# Autodesk Inventor assembly: TWambatDrive
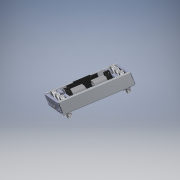
[picture p0: Inventor's stored thumbnail of the model, 180x180]
Saved by Autodesk Inventor 2019 (Build 230136000, 136)
## iProperties
Created: 2019-12-10
Part Number: TWambatDrive
Document SubType Name: Assembly
Designer: james
Author: james
## Documents named in this file (5)
- F:\JimsRobot\FIRSTRobots\Design\TWambat\TWambatDrive.iam
- F:\JimsRobot\FIRSTRobots\Design\TWambat\TWambat Side.iam
- F:\JimsRobot\FIRSTRobots\Design\TWambat\BackBatteryPlate.ipt
- F:\JimsRobot\FIRSTRobots\Design\TWambat\TWambat End Sheet.ipt
- F:\JimsRobot\FIRSTRobots\Design\TWambat\TWambat Front Sheet.ipt
## Components (6 placed, 4 different names)
1. TWambat Side:1 [sub-assembly] — Mate:1, Mate:2, Mate:3, Mate:13, Mate:14, Mate:15
2. BackBatteryPlate:1 — Mate:4, Mate:5, Mate:6, Mate:7, Mate:8, Mate:9
3. TWambat End Sheet:1 — Mate:1, Mate:2, Mate:3, Mate:4, Mate:5, Mate:6
4. TWambat End Sheet:2 — Mate:7, Mate:8, Mate:9, Mate:10, Mate:11, Mate:12
5. TWambat Side:2 [sub-assembly] — Mate:10, Mate:11, Mate:12
6. TWambat Front Sheet:1 — Mate:13, Mate:14, Mate:15
## Relationships (15: Mate 15)
- Mate:1: TWambat Side:1 ↔ TWambat End Sheet:1
- Mate:2: TWambat Side:1 ↔ TWambat End Sheet:1
- Mate:3: TWambat Side:1 ↔ TWambat End Sheet:1
- Mate:4: BackBatteryPlate:1 ↔ TWambat End Sheet:1
- Mate:5: BackBatteryPlate:1 ↔ TWambat End Sheet:1
- Mate:6: BackBatteryPlate:1 ↔ TWambat End Sheet:1
- Mate:7: BackBatteryPlate:1 ↔ TWambat End Sheet:2
- Mate:8: BackBatteryPlate:1 ↔ TWambat End Sheet:2
- Mate:9: BackBatteryPlate:1 ↔ TWambat End Sheet:2
- Mate:10: TWambat End Sheet:2 ↔ TWambat Side:2
- Mate:11: TWambat End Sheet:2 ↔ TWambat Side:2
- Mate:12: TWambat End Sheet:2 ↔ TWambat Side:2
- Mate:13: TWambat Side:1 ↔ TWambat Front Sheet:1
- Mate:14: TWambat Side:1 ↔ TWambat Front Sheet:1
- Mate:15: TWambat Side:1 ↔ TWambat Front Sheet:1
